# Autodesk Inventor assembly: 2021-2022 Grabber
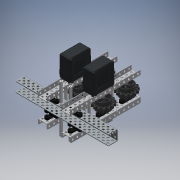
[picture p0: Inventor's stored thumbnail of the model, 180x180]
Saved by Autodesk Inventor 2019 (Build 230136000, 136)
## iProperties
Created: 2021-09-21
Part Number: 2021-2022 Grabber
Document SubType Name: Assembly
Designer: 22spencen
Author: 22spencen
## Documents named in this file (8)
- \\Chopper\2022\22spencen\Documents\VEX_CAD\Assemblies\2021-2022 Grabber.iam
- \\Chopper\2022\22spencen\Documents\VEX_CAD\Part Files\VEX Parts Library 2016\Imperial\Structure\Angle 2x2x20 Hole.ipt
- \\Chopper\2022\22spencen\Documents\VEX_CAD\Part Files\VEX Parts Library 2016\Imperial\Motion\Bearing Flat.ipt
- \\Chopper\2022\22spencen\Documents\VEX_CAD\Assemblies\2021-2022 Grabber Module.iam
- \\Chopper\2022\22spencen\Documents\VEX_CAD\Part Files\VEX Parts Library 2016\Imperial\Structure\2 inch Standoff.ipt
- \\Chopper\2022\22spencen\Documents\VEX_CAD\Part Files\VEX Parts Library 2016\Imperial\Structure\1 inch Standoff.ipt
- \\Chopper\2022\22spencen\Documents\VEX_CAD\Part Files\VEX Parts Library 2016\Imperial\Structure\0.5 inch Standoff.ipt
- U:\Svec\Robotics\Parts\Motion\V5_Smart_Motor_276-4840.iam
## Components (18 placed, 7 different names)
1. Angle 2x2x20 Hole:1 — Flush:1, Flush:2, Flush:3, Insert:2, Insert:3, Insert:10, Insert:11
2. Angle 2x2x20 Hole:2 — Flush:1, Flush:2, Flush:3, Insert:4, Insert:5, Insert:8, Insert:9
3. Bearing Flat:1 — Insert:3
4. Bearing Flat:2 — Insert:2
5. Bearing Flat:3 — Insert:4, Insert:6
6. Bearing Flat:4 — Insert:5, Insert:7
7. 2021-2022 Grabber Module:1 [sub-assembly] — Insert:6, Flush:4, Insert:13, Insert:14, Insert:17
8. 2021-2022 Grabber Module:2 [sub-assembly] — Insert:7, Flush:4, Insert:12, Insert:15, Insert:16
9. 2 inch Standoff:1 — Insert:8
10. 2 inch Standoff:2 — Insert:9
11. 2 inch Standoff:3 — Insert:10
12. 2 inch Standoff:4 — Insert:11
13. 1 inch Standoff:1 — Insert:12
14. 0.5 inch Standoff:1 — Insert:13
15. 1 inch Standoff:2 — Insert:14
16. 0.5 inch Standoff:2 — Insert:15
17. V5_Smart_Motor_276-4840:1 [sub-assembly] — Insert:17, Flush:5
18. V5_Smart_Motor_276-4840:2 [sub-assembly] — Insert:16, Flush:5
## Relationships (21: Insert 16, Flush 5)
- Flush:1: Angle 2x2x20 Hole:1 ↔ Angle 2x2x20 Hole:2
- Flush:2: Angle 2x2x20 Hole:1 ↔ Angle 2x2x20 Hole:2
- Flush:3: Angle 2x2x20 Hole:1 ↔ Angle 2x2x20 Hole:2
- Insert:2: Angle 2x2x20 Hole:1 ↔ Bearing Flat:2
- Insert:3: Angle 2x2x20 Hole:1 ↔ Bearing Flat:1
- Insert:4: Angle 2x2x20 Hole:2 ↔ Bearing Flat:3
- Insert:5: Angle 2x2x20 Hole:2 ↔ Bearing Flat:4
- Insert:6: Bearing Flat:3 ↔ 2021-2022 Grabber Module:1
- Insert:7: Bearing Flat:4 ↔ 2021-2022 Grabber Module:2
- Flush:4: 2021-2022 Grabber Module:1 ↔ 2021-2022 Grabber Module:2
- Insert:8: Angle 2x2x20 Hole:2 ↔ 2 inch Standoff:1
- Insert:9: Angle 2x2x20 Hole:2 ↔ 2 inch Standoff:2
- Insert:10: Angle 2x2x20 Hole:1 ↔ 2 inch Standoff:3
- Insert:11: Angle 2x2x20 Hole:1 ↔ 2 inch Standoff:4
- Insert:12: 2021-2022 Grabber Module:2 ↔ 1 inch Standoff:1
- Insert:13: 2021-2022 Grabber Module:1 ↔ 0.5 inch Standoff:1
- Insert:14: 2021-2022 Grabber Module:1 ↔ 1 inch Standoff:2
- Insert:15: 2021-2022 Grabber Module:2 ↔ 0.5 inch Standoff:2
- Insert:16: 2021-2022 Grabber Module:2 ↔ V5_Smart_Motor_276-4840:2
- Insert:17: 2021-2022 Grabber Module:1 ↔ V5_Smart_Motor_276-4840:1
- Flush:5: V5_Smart_Motor_276-4840:1 ↔ V5_Smart_Motor_276-4840:2
